# Autodesk Inventor assembly: ServoPlateBCoupler
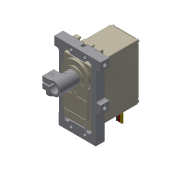
[picture p0: Inventor's stored thumbnail of the model, 180x180]
Saved by Autodesk Inventor 2018 (Build 220112000, 112)
## iProperties
Created: 2017-12-08
Part Number: ServoPlateBCoupler
Document SubType Name: Assembly
Designer: ball
Author: ball
## Documents named in this file (4)
- C:\FTC\FTC8863CAD\2017Robot\ServoPlateBCoupler.iam
- C:\FTC\FTC8863CAD\StepLibraries\HS-645 MG.ipt
- C:\FTC\FTC8863CAD\Actobotics\575 parts\575124.ipt
- C:\FTC\FTC8863CAD\Actobotics\525 parts\525148 assembly.ipt
## Components (3 placed, 3 different names)
1. HS-645 MG:1 — Mate:1, Mate:2, Mate:3, Mate:4, Mate:5
2. 575124:1 — Mate:1, Mate:2, Mate:3
3. 525148 assembly:1 — Mate:4, Mate:5
## Relationships (5: Mate 5)
- Mate:1: HS-645 MG:1 ↔ 575124:1
- Mate:2: HS-645 MG:1 ↔ 575124:1
- Mate:3: HS-645 MG:1 ↔ 575124:1
- Mate:4: HS-645 MG:1 ↔ 525148 assembly:1
- Mate:5: HS-645 MG:1 ↔ 525148 assembly:1
